# Autodesk Inventor assembly: Origami Printer
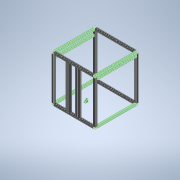
[picture p0: Inventor's stored thumbnail of the model, 180x180]
Saved by Autodesk Inventor 2022 (Build 260153000, 153)
## iProperties
Created: 2021-10-05
Part Number: Origami Printer
Document SubType Name: Assembly
Designer: nicol
Author: nicol
## iProperties of the stored document MemberDocs/xI5wsq5txEsj0qh4kHnbhpr4qBb
Created: 2021-10-05
Part Number: Origami Printer
Document SubType Name: Assembly
Designer: nicol
Author: nicol
## Documents named in this file (17)
- C:\Users\nicol\Documents\_Origami Printer\Origami Printer.iam
- C:\Users\nicol\Documents\_Origami Printer\2020 Extrusions\2020 X Axis.ipt
- C:\Users\nicol\Documents\_Origami Printer\2020 Extrusions\2020 Y Axis.ipt
- C:\Users\nicol\Documents\_Origami Printer\2020 Extrusions\2020 Z Axis.ipt
- C:\Users\nicol\Documents\_Origami Printer\2020 Extrusions\2040 Z Axis Upright.ipt
- C:\Users\nicol\Documents\_Origami Printer\2020 Extrusions\Corner Connector.ipt
- C:\Users\nicol\Documents\_Origami Printer\2020 Extrusions\Corner Cube.ipt
- C:\Users\nicol\Documents\_Origami Printer\Sheet Metal\Z Drive Mount v7.ipt
- C:\Users\nicol\Documents\_Origami Printer\Electronics\NEMA 17.ipt
- C:\Users\nicol\Documents\_Origami Printer\3D printed\Z Drive Bearing Holder.ipt
- C:\Users\nicol\Documents\_Origami Printer\Bearings\625 Bearing.ipt
- C:\Users\nicol\Documents\_Origami Printer\Hardware\5 x 50mm Shaft.ipt
- C:\Users\nicol\Documents\_Origami Printer\Hardware\GT2 Pulley 16T.ipt
- C:\Users\nicol\Documents\_Origami Printer\Hardware\METAL WORM GEAR_57545K624 v5.ipt
- C:\Users\nicol\Documents\_Origami Printer\Hardware\PLASTIC WORM GEAR_4037N115 v3.ipt
- C:\Users\nicol\Documents\_Origami Printer\Hardware\MGN-12H.iam
- C:\Users\nicol\Documents\_Origami Printer\Sheet Metal\X Axis Cross v10.ipt
## Components (26 placed, 7 different names)
1. 2020 X Axis:1 — Insert:13, Insert:17
2. 2020 Y Axis:1 — Insert:22
3. 2020 Z Axis:1 — Insert:20, Insert:21, Mate:3
4. 2040 Z Axis Upright:1 — Flush:1, Mate:7, Mate:10, Flush:5, Flush:6
5. Corner Connector:1
6. Corner Cube:1 — Insert:11, Insert:12, Insert:13
7. 2040 Z Axis Upright:2 — Flush:1, Mate:6, Mate:9
8. 2020 Z Axis:2 — Insert:1, Insert:2, Mate:1, Mate:2
9. 2020 Z Axis:3 — Insert:6, Insert:11
10. 2020 Z Axis:4 — Insert:18, Insert:19
11. 2020 Y Axis:2 — Mate:3
12. 2020 Y Axis:3 — Insert:23
13. 2020 Y Axis:4 — Insert:5, Mate:2, Insert:7
14. 2020 X Axis:2 — Insert:10, Insert:16, Flush:4, Mate:8
15. 2020 X Axis:3 — Insert:9, Insert:14, Mate:6, Mate:7, Flush:4, Flush:6
16. 2020 X Axis:4 — Insert:8, Insert:15
17. 2020 Y Axis:5 — Insert:4, Insert:12
18. 2020 Y Axis:6 — Mate:1
19. Corner Cube:2 — Insert:6, Insert:7, Insert:8
20. Corner Cube:3 — Insert:2, Insert:4, Insert:10
21. Corner Cube:4 — Insert:1, Insert:5, Insert:9
22. Corner Cube:5 — Insert:14, Insert:19
23. Corner Cube:6 — Insert:15, Insert:20, Insert:23
24. Corner Cube:7 — Insert:16, Insert:18
25. Corner Cube:8 — Insert:17, Insert:21, Insert:22
26. Z Drive Mount v7:1 — Mate:8, Mate:9, Mate:10, Flush:5
## Relationships (34: Insert 22, Mate 8, Flush 4)
- Insert:1: 2020 Z Axis:2 ↔ Corner Cube:4
- Insert:2: 2020 Z Axis:2 ↔ Corner Cube:3
- Insert:4: 2020 Y Axis:5 ↔ Corner Cube:3
- Insert:5: 2020 Y Axis:4 ↔ Corner Cube:4
- Mate:1: 2020 Z Axis:2 ↔ 2020 Y Axis:6
- Mate:2: 2020 Z Axis:2 ↔ 2020 Y Axis:4
- Insert:6: 2020 Z Axis:3 ↔ Corner Cube:2
- Insert:7: 2020 Y Axis:4 ↔ Corner Cube:2
- Insert:8: 2020 X Axis:4 ↔ Corner Cube:2
- Insert:9: 2020 X Axis:3 ↔ Corner Cube:4
- Insert:10: 2020 X Axis:2 ↔ Corner Cube:3
- Insert:11: Corner Cube:1 ↔ 2020 Z Axis:3
- Insert:12: Corner Cube:1 ↔ 2020 Y Axis:5
- Insert:13: 2020 X Axis:1 ↔ Corner Cube:1
- Insert:14: 2020 X Axis:3 ↔ Corner Cube:5
- Insert:15: 2020 X Axis:4 ↔ Corner Cube:6
- Insert:16: 2020 X Axis:2 ↔ Corner Cube:7
- Insert:17: 2020 X Axis:1 ↔ Corner Cube:8
- Insert:18: 2020 Z Axis:4 ↔ Corner Cube:7
- Insert:19: 2020 Z Axis:4 ↔ Corner Cube:5
- Insert:20: 2020 Z Axis:1 ↔ Corner Cube:6
- Insert:21: 2020 Z Axis:1 ↔ Corner Cube:8
- Insert:22: 2020 Y Axis:1 ↔ Corner Cube:8
- Insert:23: 2020 Y Axis:3 ↔ Corner Cube:6
- Mate:3: 2020 Z Axis:1 ↔ 2020 Y Axis:2
- Flush:1: 2040 Z Axis Upright:1 ↔ 2040 Z Axis Upright:2
- Mate:6: 2040 Z Axis Upright:2 ↔ 2020 X Axis:3
- Mate:7: 2040 Z Axis Upright:1 ↔ 2020 X Axis:3
- Flush:4: 2020 X Axis:2 ↔ 2020 X Axis:3
- Mate:8: 2020 X Axis:2 ↔ Z Drive Mount v7:1
- Mate:9: 2040 Z Axis Upright:2 ↔ Z Drive Mount v7:1
- Mate:10: 2040 Z Axis Upright:1 ↔ Z Drive Mount v7:1
- Flush:5: 2040 Z Axis Upright:1 ↔ Z Drive Mount v7:1
- Flush:6: 2040 Z Axis Upright:1 ↔ 2020 X Axis:3
